# Autodesk Inventor assembly: MotorMountAssem
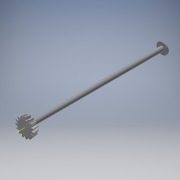
[picture p0: Inventor's stored thumbnail of the model, 180x180]
Saved by Autodesk Inventor 2017 (Build 210142000, 142)
## iProperties
Created: 2016-12-23
Part Number: MotorMountAssem
Document SubType Name: Assembly
Designer: David Kopala
Author: David Kopala
## Documents named in this file (3)
- \\Mac\Home\Documents\Drone\Drone\3D Models\Project\Chasis_02\MotorMountAssem.iam
- \\Mac\Home\Documents\Drone\Drone\3D Models\Project\Chasis_02\MotorMount.ipt
- \\Mac\Home\Documents\Drone\Drone\3D Models\Project\Chasis_02\Bottom_Bevel_Driver.ipt
## Components (2 placed, 2 different names)
1. MotorMount:1 — Insert:1
2. Bevel Gear2:1 — Insert:1
## Relationships (1: Insert 1)
- Insert:1: MotorMount:1 ↔ Bevel Gear2:1
